# Autodesk Inventor assembly: Сборка7
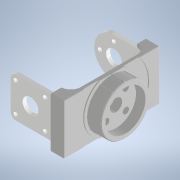
[picture p0: Inventor's stored thumbnail of the model, 180x180]
Saved by Autodesk Inventor 2022 (Build 260153000, 153)
## iProperties
Created: 2023-02-13
Part Number: Сборка7
Document SubType Name: Assembly
Designer: Папа
Author: Папа
## Documents named in this file (3)
- E:\Новая папка\Сборка7.iam
- E:\Новая папка\мотор_локтя_2+П.ipt
- E:\Новая папка\ZJ-DUAN.ipt
## Components (2 placed, 2 different names)
1. мотор_локтя_2+П:1 — Совмещение:1, Совмещение:2, Совмещение:3
2. ZJ-DUAN:1 — Совмещение:1, Совмещение:2, Совмещение:3
## Relationships (3: Mate 3)
- Совмещение:1 [Mate]: мотор_локтя_2+П:1 ↔ ZJ-DUAN:1
- Совмещение:2 [Mate]: мотор_локтя_2+П:1 ↔ ZJ-DUAN:1
- Совмещение:3 [Mate]: мотор_локтя_2+П:1 ↔ ZJ-DUAN:1
